# Autodesk Inventor assembly: DoubleCrossRail
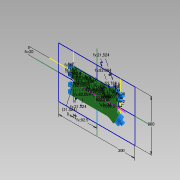
[picture p0: Inventor's stored thumbnail of the model, 180x180]
Saved by Autodesk Inventor 2021 (Build 250183000, 183)
## iProperties
Created: 2021-02-18
Part Number: DoubleCrossRail
Document SubType Name: Assembly
Designer: kumagai
Author: kumagai
## Documents named in this file (4)
- X:\Develop\CAD\PlaRails\DoubleCross\DoubleCrossRail.iam
- X:\Develop\CAD\PlaRails\RailJointFemale.ipt
- X:\Develop\CAD\PlaRails\RailJointMale.ipt
- X:\Develop\CAD\PlaRails\DoubleCross\DoubleCross.ipt
## Components (5 placed, 3 different names)
1. DoubleCross:1 — フラッシュ:1, フラッシュ:2, フラッシュ:3, フラッシュ:4, フラッシュ:5, フラッシュ:6, フラッシュ:7, フラッシュ:8, メイト:1, メイト:2, メイト:3, メイト:4
2. RailJointFemale:1 — フラッシュ:5, フラッシュ:8, メイト:1
3. RailJointFemale:2 — フラッシュ:6, フラッシュ:7, メイト:2
4. RailJointMale:1 — フラッシュ:2, フラッシュ:4, メイト:3
5. RailJointMale:2 — フラッシュ:1, フラッシュ:3, メイト:4
## Relationships (12: Flush 8, Mate 4)
- フラッシュ:1 [Flush]: DoubleCross:1 ↔ RailJointMale:2
- フラッシュ:2 [Flush]: DoubleCross:1 ↔ RailJointMale:1
- フラッシュ:3 [Flush]: DoubleCross:1 ↔ RailJointMale:2
- フラッシュ:4 [Flush]: DoubleCross:1 ↔ RailJointMale:1
- フラッシュ:5 [Flush]: DoubleCross:1 ↔ RailJointFemale:1
- フラッシュ:6 [Flush]: DoubleCross:1 ↔ RailJointFemale:2
- フラッシュ:7 [Flush]: DoubleCross:1 ↔ RailJointFemale:2
- フラッシュ:8 [Flush]: DoubleCross:1 ↔ RailJointFemale:1
- メイト:1 [Mate]: DoubleCross:1 ↔ RailJointFemale:1
- メイト:2 [Mate]: DoubleCross:1 ↔ RailJointFemale:2
- メイト:3 [Mate]: DoubleCross:1 ↔ RailJointMale:1
- メイト:4 [Mate]: DoubleCross:1 ↔ RailJointMale:2
